# Autodesk Inventor assembly: Double Sprocket Axle
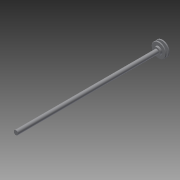
[picture p0: Inventor's stored thumbnail of the model, 180x180]
Saved by Autodesk Inventor 2015 (Build 190159000, 159)
## iProperties
Created: 2015-01-11
Part Number: Double Sprocket Axle
Document SubType Name: Assembly
Designer: chapale16
Author: chapale16
## Documents named in this file (3)
- \\lhssvr02\Homedirs\Robotics Club\CAD Model 2015\Box Beam Drive Base\Double Sprocket Axle.iam
- \\lhssvr02\Homedirs\Robotics Club\CAD Model 2015\Box Beam Drive Base\Conveyor Axle.ipt
- H:\Sprocket Large.ipt
## Components (3 placed, 2 different names)
1. Conveyor Axle:1 — Mate:1, Mate:2
2. Sprocket Large:2 — Mate:1
3. Sprocket Large:3 — Mate:2
## Relationships (2: Mate 2)
- Mate:1: Conveyor Axle:1 ↔ Sprocket Large:2
- Mate:2: Conveyor Axle:1 ↔ Sprocket Large:3
